# Autodesk Inventor assembly: SiCMonoFilamentMicroheaterPrintHead_LessHeatSinks
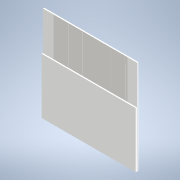
[picture p0: Inventor's stored thumbnail of the model, 180x180]
Saved by Autodesk Inventor 2021 (Build 250183000, 183)
## iProperties
Created: 2021-10-17
Part Number: SiCMonoFilamentMicroheaterPrintHead_LessHeatSinks
Document SubType Name: Assembly
Designer: Unit-005
Author: Unit-005
## Documents named in this file (5)
- C:\Users\Unit-005\Documents\Inventor\SiC_Monofilament_MicroheaterPrinthead\SiCMonoFilamentMicroheaterPrintHead_LessHeatSinks.iam
- C:\Users\Unit-005\Documents\Inventor\SiC_Monofilament_MicroheaterPrinthead\Al2O3PowerSideSubstrate.ipt
- C:\Users\Unit-005\Documents\Inventor\SiC_Monofilament_MicroheaterPrinthead\Leads.ipt
- C:\Users\Unit-005\Documents\Inventor\SiC_Monofilament_MicroheaterPrinthead\SiCElement.ipt
- C:\Users\Unit-005\Documents\Inventor\SiC_Monofilament_MicroheaterPrinthead\ContactPlate.ipt
## Components (4 placed, 4 different names)
1. Al2O3PowerSideSubstrate:1 — Mate:2, Flush:1, Mate:3, Mate:5
2. Leads:1 — Mate:2, Flush:1, Mate:3, Mate:4, Mate:7
3. SiCElement:1 — Mate:4, Mate:5, Flush:2, Mate:6, Mate:7, Mate:8
4. ContactPlate:1 — Flush:2, Mate:6, Mate:8
## Relationships (9: Mate 7, Flush 2)
- Mate:2: Al2O3PowerSideSubstrate:1 ↔ Leads:1
- Flush:1: Al2O3PowerSideSubstrate:1 ↔ Leads:1
- Mate:3: Al2O3PowerSideSubstrate:1 ↔ Leads:1
- Mate:4 (0.0675 mm): Leads:1 ↔ SiCElement:1
- Mate:5 (-0.0675 mm): Al2O3PowerSideSubstrate:1 ↔ SiCElement:1
- Flush:2 (0.0675 mm): SiCElement:1 ↔ ContactPlate:1
- Mate:6 (-0.0675 mm): SiCElement:1 ↔ ContactPlate:1
- Mate:7: Leads:1 ↔ SiCElement:1
- Mate:8: SiCElement:1 ↔ ContactPlate:1
